# Autodesk Inventor assembly: Box
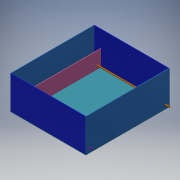
[picture p0: Inventor's stored thumbnail of the model, 180x180]
Saved by Autodesk Inventor 2017 (Build 210142000, 142)
## iProperties
Created: 2017-11-22
Part Number: Box
Document SubType Name: Assembly
Designer: guirguk
Author: guirguk
## Documents named in this file (7)
- C:\Users\guirguk\Documents\LazyBots\Box.iam
- C:\Users\guirguk\Documents\LazyBots\Base.ipt
- C:\Users\guirguk\Documents\LazyBots\Front.ipt
- C:\Users\guirguk\Documents\LazyBots\Side.ipt
- C:\Users\guirguk\Documents\LazyBots\inner_wall.ipt
- C:\Users\guirguk\Documents\LazyBots\Long_Shaft.ipt
- C:\Users\guirguk\Documents\LazyBots\Short_Shaft.ipt
## Components (10 placed, 6 different names)
1. Base:1 — Flush:1, Mate:1, Flush:2, Flush:3, Mate:2, Flush:4, Mate:4, Mate:6, Mate:8, Mate:11
2. Side:1 — Flush:1, Mate:1, Flush:2, Flush:5, Mate:3, Flush:6, Mate:9, Flush:7
3. Side:2 — Flush:3, Mate:2, Flush:4, Mate:5, Mate:12
4. Front:1 — Flush:5, Mate:3, Mate:4, Mate:7, Mate:10
5. Front:2 — Flush:6, Mate:5, Mate:6
6. inner_wall:1 — Mate:7, Mate:8, Mate:9, Tangent:3, Flush:9
7. inner_wall:2 — Mate:10, Mate:11, Mate:12, Tangent:1, Tangent:2, Flush:8
8. Long_Shaft:1 — Tangent:1, Flush:7
9. Short_Shaft:1 — Tangent:2, Flush:8
10. Short_Shaft:2 — Tangent:3, Flush:9
## Relationships (24: Mate 12, Flush 9, Tangent 3)
- Flush:1: Base:1 ↔ Side:1
- Mate:1: Base:1 ↔ Side:1
- Flush:2: Base:1 ↔ Side:1
- Flush:3: Base:1 ↔ Side:2
- Mate:2: Base:1 ↔ Side:2
- Flush:4: Base:1 ↔ Side:2
- Flush:5: Side:1 ↔ Front:1
- Mate:3: Side:1 ↔ Front:1
- Mate:4: Base:1 ↔ Front:1
- Flush:6: Side:1 ↔ Front:2
- Mate:5: Side:2 ↔ Front:2
- Mate:6: Base:1 ↔ Front:2
- Mate:7: Front:1 ↔ inner_wall:1
- Mate:8: Base:1 ↔ inner_wall:1
- Mate:9 (38.1 mm): Side:1 ↔ inner_wall:1
- Mate:10: Front:1 ↔ inner_wall:2
- Mate:11: Base:1 ↔ inner_wall:2
- Mate:12 (38.1 mm): Side:2 ↔ inner_wall:2
- Tangent:1: inner_wall:2 ↔ Long_Shaft:1
- Flush:7 (-25.4 mm): Side:1 ↔ Long_Shaft:1
- Tangent:2: inner_wall:2 ↔ Short_Shaft:1
- Flush:8: inner_wall:2 ↔ Short_Shaft:1
- Tangent:3: inner_wall:1 ↔ Short_Shaft:2
- Flush:9: inner_wall:1 ↔ Short_Shaft:2
